# Autodesk Inventor assembly: MechanumChassis
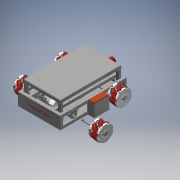
[picture p0: Inventor's stored thumbnail of the model, 180x180]
Saved by Autodesk Inventor 2018 (Build 220112000, 112)
## iProperties
Created: 2017-10-18
Part Number: MechanumChassis
Document SubType Name: Weldment
Designer: Bryce Richards
Mass: 42172.1 g
Surface Area: 44852.8 cm^2
Volume: 5448.29 cm^3
Density: 7.74044 g/cm^3
Weld Material: Steel, Mild, Welded
Author: Bryce Richards
## Documents named in this file (35)
- C:\Users\P136265\Documents\GitHub\mecanum-cad\MechanumChassis.iam
- C:\Users\P136265\Documents\GitHub\mecanum-cad\MecanumFrame2.iam
- C:\Users\P136265\Documents\GitHub\mecanum-cad\PillowAssembly.iam
- C:\Users\P136265\Documents\Inventor\Content Center Files\R2018\en-US\AS 1110\AS 1110 - M8 x 60.ipt
- C:\Users\P136265\Documents\Inventor\Content Center Files\R2018\en-US\AS 1112 (2)\AS 1112 - M8  Type 5.ipt
- C:\Users\P136265\Documents\GitHub\mecanum-cad\PillowPlate.ipt
- C:\Users\P136265\Documents\GitHub\mecanum-cad\LiftPlate.iam
- C:\Users\P136265\Documents\GitHub\mecanum-cad\AlignmentTube.ipt
- C:\Users\P136265\Documents\GitHub\mecanum-cad\WheelShaft.ipt
- C:\Users\P136265\Documents\GitHub\mecanum-cad\Mecanum_Assembly.iam
- C:\Users\P136265\Documents\Inventor\Content Center Files\R2018\en-US\ISO 4032(2)\ISO 4032 - M20 - ISO.ipt
- C:\Users\P136265\Documents\GitHub\mecanum-cad\Cover_FrontRear.ipt
- C:\Users\P136265\Documents\Inventor\Content Center Files\R2018\en-US\CNS 4373\CNS 4373 - M 4.ipt
- C:\Users\P136265\Documents\GitHub\mecanum-cad\Cover_LiftSurface.ipt
- C:\Users\P136265\Documents\GitHub\mecanum-cad\Compressor_PX06.ipt
- C:\Users\P136265\Documents\GitHub\mecanum-cad\RestraintPlate.ipt
- C:\Users\P136265\Documents\Inventor\Content Center Files\R2018\en-US\AS 1420\AS 1420 - 1973 - M4 x 12.ipt
- C:\Users\P136265\Documents\GitHub\mecanum-cad\Cover_Rear.ipt
- C:\Users\P136265\Documents\Inventor\Content Center Files\R2018\en-US\AS 1112 (2)\AS 1112 - M4  Type 5.ipt
- C:\Users\P136265\Documents\Inventor\Content Center Files\R2018\en-US\AS 1110\AS 1110 - M4 x 10.ipt
- C:\Users\P136265\Documents\GitHub\mecanum-cad\LiftBase.ipt
- C:\Users\P136265\Documents\GitHub\mecanum-cad\Firestone.ipt
- C:\Users\P136265\Documents\Inventor\Content Center Files\R2018\en-US\AS 1110\AS 1110 - M8 x 12.ipt
- C:\Users\P136265\Documents\GitHub\mecanum-cad\Nema 23 Stepper Motor Bipolar L=56mm w Gear Ratio 41 Planetary Gearbox.ipt
- C:\Users\P136265\Documents\GitHub\mecanum-cad\Cover_Left.ipt
- C:\Users\P136265\Documents\GitHub\mecanum-cad\Cover_Right.ipt
- C:\Users\P136265\Documents\GitHub\mecanum-cad\BatteryBox_NP1812.ipt
- C:\Users\P136265\Documents\GitHub\mecanum-cad\NP18-12 Battery.ipt
- C:\Users\P136265\Documents\GitHub\mecanum-cad\BearingHousing.iam
- C:\Users\P136265\Documents\mecanum-cad\MechanumChassis\AIP\FEA\cayefugld.fres
- C:\Users\P136265\Documents\mecanum-cad\MechanumChassis\AIP\FEA\cayefugao.fins
- C:\Users\P136265\Documents\mecanum-cad\MechanumChassis\AIP\FEA\cayefugao.fsat
- C:\Users\P136265\Documents\mecanum-cad\MechanumChassis\AIP\FEA\cayefugao.ftes
- C:\Users\P136265\Documents\mecanum-cad\MechanumChassis\AIP\FEA\cayefugao.fwiz
- C:\Users\P136265\Documents\mecanum-cad\MechanumChassis\AIP\FEA\cayefuglc.fmsh
## Components (143 placed, 28 different names)
1. MecanumFrame2:1 [sub-assembly] — Flush:2, Flush:6, Mate:69, Mate:70, Mate:71, Mate:90, Angle:5, Angle:6, Angle:7, Flush:10, Insert:17, Insert:18, Insert:19, Insert:20, Insert:21, Insert:22, Insert:23, Insert:24, Insert:25, Insert:26, Insert:27, Insert:28, Insert:29, Insert:30, Insert:31, Insert:32, Angle:8, Mate:209, Mate:210, Flush:11, Angle:9, Angle:10, Angle:11, Mate:211, Mate:212, Flush:12, Mate:213, Mate:214, Flush:13, Mate:215, Mate:216, Flush:14, Mate:234, Mate:235, Mate:236, Angle:29, Mate:263, Mate:283, Mate:285, Mate:287, Mate:289, Mate:303, Mate:305, Mate:307, Mate:309, Mate:353, Mate:354, Mate:355, Mate:386, Flush:32, Flush:33, Angle:34, Mate:410, Mate:411, Mate:412, Mate:413, Mate:414, Mate:415, Mate:416, Mate:417, Mate:418, Mate:419, Mate:420, Mate:421, Mate:423, Mate:425, Mate:427, Mate:429, Mate:431, Mate:433, Mate:435, Mate:437, Mate:439, Mate:441, Mate:443, Mate:445, Mate:447, Mate:449, Mate:451, Mate:482, Mate:483, Mate:484
2. PillowAssembly:1 [sub-assembly] — Mate:16, Mate:59, Mate:186, Mate:190, Mate:234
3. PillowAssembly:2 [sub-assembly] — Mate:13, Mate:62, Mate:178, Mate:180, Mate:235
4. PillowAssembly:3 [sub-assembly] — Mate:15, Mate:63, Mate:64, Mate:202, Mate:206, Mate:236
5. PillowAssembly:5 [sub-assembly] — Mate:13, Flush:2, Mate:60, Mate:61, Mate:182, Mate:184, Mate:320, Flush:29, Mate:329
6. PillowAssembly:6 [sub-assembly] — Mate:15, Mate:65, Flush:10, Mate:204, Mate:208, Mate:317, Flush:27, Mate:327
7. PillowAssembly:7 [sub-assembly] — Flush:6, Mate:16, Mate:57, Mate:58, Mate:188, Mate:192, Mate:323, Flush:31, Mate:331
8. PillowPlate:2 — Mate:57, Mate:58, Mate:59, Mate:71
9. PillowPlate:3 — Mate:60, Mate:61, Mate:62, Mate:70
10. PillowPlate:4 — Mate:63, Mate:64, Mate:65, Mate:69
11. LiftPlate:1 [sub-assembly] — Angle:29, Angle:30, Angle:31, Angle:32, Angle:33, Mate:263, Mate:311, Flush:22, Flush:23, Mate:413, Mate:414, Mate:481
12. AS 1110 - Metric M8 x 60:33 — Insert:17, Mate:179
13. AS 1110 - Metric M8 x 60:34 — Insert:18, Mate:177
14. AS 1110 - Metric M8 x 60:35 — Insert:19, Mate:183
15. AS 1110 - Metric M8 x 60:36 — Insert:20, Mate:181
16. AS 1110 - Metric M8 x 60:37 — Insert:21, Mate:187
17. AS 1110 - Metric M8 x 60:38 — Insert:22, Mate:191
18. AS 1110 - Metric M8 x 60:39 — Insert:23, Mate:189
19. AS 1110 - Metric M8 x 60:40 — Insert:24, Mate:185
20. AS 1110 - Metric M8 x 60:41 — Insert:25, Mate:199
21. AS 1110 - Metric M8 x 60:42 — Insert:26, Mate:197
22. AS 1110 - Metric M8 x 60:43 — Insert:27, Mate:195
23. AS 1110 - Metric M8 x 60:44 — Insert:28, Mate:193
24. AS 1110 - Metric M8 x 60:45 — Insert:29, Mate:201
25. AS 1110 - Metric M8 x 60:46 — Insert:30, Mate:203
26. AS 1110 - Metric M8 x 60:47 — Insert:31, Mate:207
27. AS 1110 - Metric M8 x 60:48 — Insert:32, Mate:205
28. AS 1112 (2) - Metric M8  Type 5:33 — Mate:177, Mate:178
29. AS 1112 (2) - Metric M8  Type 5:34 — Mate:179, Mate:180
30. AS 1112 (2) - Metric M8  Type 5:35 — Mate:181, Mate:182
31. AS 1112 (2) - Metric M8  Type 5:36 — Mate:183, Mate:184
32. AS 1112 (2) - Metric M8  Type 5:37 — Mate:185, Mate:186
33. AS 1112 (2) - Metric M8  Type 5:38 — Mate:187, Mate:188
34. AS 1112 (2) - Metric M8  Type 5:39 — Mate:189, Mate:190
35. AS 1112 (2) - Metric M8  Type 5:40 — Mate:191, Mate:192
36. AS 1112 (2) - Metric M8  Type 5:41 — Mate:193
37. AS 1112 (2) - Metric M8  Type 5:42 — Mate:195
38. AS 1112 (2) - Metric M8  Type 5:43 — Mate:197
39. AS 1112 (2) - Metric M8  Type 5:44 — Mate:199
40. AS 1112 (2) - Metric M8  Type 5:45 — Mate:201, Mate:202
41. AS 1112 (2) - Metric M8  Type 5:46 — Mate:203, Mate:204
42. AS 1112 (2) - Metric M8  Type 5:47 — Mate:205, Mate:206
43. AS 1112 (2) - Metric M8  Type 5:48 — Mate:207, Mate:208
44. AlignmentTube:1 — Angle:10, Mate:213, Mate:214, Flush:13, Angle:33
45. AlignmentTube:2 — Angle:8, Mate:209, Mate:210, Flush:11, Angle:31
46. AlignmentTube:3 — Angle:11, Mate:215, Mate:216, Flush:14, Angle:32
47. AlignmentTube:4 — Angle:9, Mate:211, Mate:212, Flush:12, Angle:30
48. Mecanum_Assembly:1 [sub-assembly] — Mate:318, Mate:319, Flush:28, Mate:344, Mate:345, Mate:346, Mate:351
49. Mecanum_Assembly:2 [sub-assembly] — Mate:321, Mate:322, Flush:30, Mate:341, Mate:342, Mate:343, Mate:349
50. Mecanum_Assembly:3 [sub-assembly] — Mate:315, Mate:316, Flush:26, Mate:338, Mate:339, Mate:340, Mate:347
51. Mecanum_Assembly:4 [sub-assembly] — Mate:312, Flush:24, Mate:314, Mate:333, Mate:334, Mate:335, Mate:336
52. Cover_FrontRear:1 — Mate:410, Mate:411, Mate:412
53. CNS 4373 M 4:7 — Mate:283
54. CNS 4373 M 4:8 — Mate:285
55. CNS 4373 M 4:9 — Mate:287
56. CNS 4373 M 4:10 — Mate:289
57. CNS 4373 M 4:17 — Mate:303
58. CNS 4373 M 4:18 — Mate:305
59. CNS 4373 M 4:19 — Mate:307
60. CNS 4373 M 4:20 — Mate:309
61. Cover_LiftSurface:1 — Mate:311, Flush:22, Flush:23
62. WheelShaft:1 — Mate:312, Flush:24, Mate:314, Mate:324, Mate:485
63. WheelShaft:2 — Mate:318, Mate:319, Flush:28, Mate:320, Flush:29, Mate:328
64. WheelShaft:3 — Mate:315, Mate:316, Flush:26, Mate:317, Flush:27, Mate:326
65. WheelShaft:4 — Mate:321, Mate:322, Flush:30, Mate:323, Flush:31, Mate:330, Mate:394
66. ISO 4032 M20:1 — Mate:324
67. ISO 4032 M20:2 — Mate:326, Mate:327
68. ISO 4032 M20:3 — Mate:328, Mate:329
69. ISO 4032 M20:4 — Mate:330, Mate:331
70. Compressor_PX06:1 — Mate:356, Mate:358, Mate:367, Mate:368, Mate:369, Mate:370, Mate:371, Mate:372, Mate:373, Mate:374, Mate:375, Mate:376, Mate:377
71. RestraintPlate:1 — Mate:333, Mate:334, Mate:335, Mate:337
72. RestraintPlate:2 — Mate:338, Mate:339, Mate:340, Mate:348
73. RestraintPlate:3 — Mate:341, Mate:342, Mate:343, Mate:350
74. RestraintPlate:4 — Mate:344, Mate:345, Mate:346, Mate:352
75. Cover_Rear:1 — Mate:353, Mate:354, Mate:355, Mate:356, Mate:358, Mate:367, Mate:368, Mate:369, Mate:379, Mate:381, Mate:383, Mate:385
76. AS 1110 - Metric M4 x 10:1 — Mate:370, Mate:371, Mate:378
77. AS 1110 - Metric M4 x 10:2 — Mate:372, Mate:373, Mate:384
78. AS 1110 - Metric M4 x 10:3 — Mate:374, Mate:375, Mate:380
79. AS 1110 - Metric M4 x 10:4 — Mate:376, Mate:377, Mate:382
80. AS 1112 (2) - Metric M4  Type 5:1 — Mate:378, Mate:379
81. AS 1112 (2) - Metric M4  Type 5:2 — Mate:380, Mate:381
82. AS 1112 (2) - Metric M4  Type 5:3 — Mate:382, Mate:383
83. AS 1112 (2) - Metric M4  Type 5:4 — Mate:384, Mate:385
84. LiftBase:1 — Mate:386, Flush:32, Flush:33, Mate:387, Mate:388, Mate:389, Mate:391, Mate:393
85. Firestone:1 — Mate:387, Mate:388, Mate:389, Mate:390, Mate:392, Mate:481
86. AS 1110 - Metric M8 x 12:1 — Mate:390, Mate:391
87. AS 1110 - Metric M8 x 12:2 — Mate:392, Mate:393
88. Nema 23 Stepper Motor Bipolar L=56mm w Gear Ratio 41 Planetary Gearbox:1 — Angle:34, Mate:394
89. Cover_Left:1 — Mate:415, Mate:416, Mate:417, Mate:422, Mate:424, Mate:426, Mate:428, Mate:430, Mate:432, Mate:434, Mate:436, Mate:453, Mate:454, Mate:455, Mate:460, Mate:465, Mate:467, Mate:469, Mate:471
90. Cover_Right:1 — Mate:418, Mate:419, Mate:420, Mate:438, Mate:440, Mate:442, Mate:444, Mate:446, Mate:448, Mate:450, Mate:452, Mate:456, Mate:457, Mate:458, Mate:463, Mate:473, Mate:475, Mate:477, Mate:479
91. CNS 4373 M 4:21 — Mate:421, Mate:422
92. CNS 4373 M 4:22 — Mate:423, Mate:424
93. CNS 4373 M 4:23 — Mate:425, Mate:426
94. CNS 4373 M 4:24 — Mate:427, Mate:428
95. CNS 4373 M 4:25 — Mate:429, Mate:430
96. CNS 4373 M 4:26 — Mate:431, Mate:432
97. CNS 4373 M 4:27 — Mate:433, Mate:434
98. CNS 4373 M 4:28 — Mate:435, Mate:436
99. CNS 4373 M 4:29 — Mate:437, Mate:438
100. CNS 4373 M 4:30 — Mate:439, Mate:440
101. CNS 4373 M 4:31 — Mate:441, Mate:442
102. CNS 4373 M 4:32 — Mate:443, Mate:444
103. CNS 4373 M 4:33 — Mate:445, Mate:446
104. CNS 4373 M 4:34 — Mate:447, Mate:448
105. CNS 4373 M 4:35 — Mate:449, Mate:450
106. CNS 4373 M 4:36 — Mate:451, Mate:452
107. BatteryBox_NP1812:1 — Mate:453, Mate:454, Mate:455, Mate:459, Mate:461, Mate:466, Mate:468, Mate:470, Mate:472
108. BatteryBox_NP1812:2 — Mate:456, Mate:457, Mate:458, Mate:462, Mate:464, Mate:474, Mate:476, Mate:478, Mate:480
109. NP18-12 Battery:1 — Mate:459, Mate:460, Mate:461
110. NP18-12 Battery:2 — Mate:462, Mate:463, Mate:464
111. AS 1112 (2) - Metric M4  Type 5:5 — Mate:465, Mate:466
112. AS 1112 (2) - Metric M4  Type 5:6 — Mate:467, Mate:468
113. AS 1112 (2) - Metric M4  Type 5:7 — Mate:469, Mate:470
114. AS 1112 (2) - Metric M4  Type 5:8 — Mate:471, Mate:472
115. AS 1112 (2) - Metric M4  Type 5:9 — Mate:473, Mate:474
116. AS 1112 (2) - Metric M4  Type 5:10 — Mate:475, Mate:476
117. AS 1112 (2) - Metric M4  Type 5:11 — Mate:477, Mate:478
118. AS 1112 (2) - Metric M4  Type 5:12 — Mate:479, Mate:480
119. BearingHousing:1 [sub-assembly] — Mate:482, Mate:483, Mate:484, Mate:485
120. AS 1420 - Metric M4 x 12:1 — Mate:336, Mate:337
121. AS 1420 - Metric M4 x 12:2
122. AS 1420 - Metric M4 x 12:3
123. AS 1420 - Metric M4 x 12:4
124. AS 1420 - Metric M4 x 12:5
125. AS 1420 - Metric M4 x 12:6
126. AS 1420 - Metric M4 x 12:7 — Mate:347, Mate:348
127. AS 1420 - Metric M4 x 12:8
128. AS 1420 - Metric M4 x 12:9
129. AS 1420 - Metric M4 x 12:10
130. AS 1420 - Metric M4 x 12:11
131. AS 1420 - Metric M4 x 12:12
132. AS 1420 - Metric M4 x 12:13 — Mate:349, Mate:350
133. AS 1420 - Metric M4 x 12:14
134. AS 1420 - Metric M4 x 12:15
135. AS 1420 - Metric M4 x 12:16
136. AS 1420 - Metric M4 x 12:17
137. AS 1420 - Metric M4 x 12:18
138. AS 1420 - Metric M4 x 12:19 — Mate:351, Mate:352
139. AS 1420 - Metric M4 x 12:20
140. AS 1420 - Metric M4 x 12:21
141. AS 1420 - Metric M4 x 12:22
142. AS 1420 - Metric M4 x 12:23
143. AS 1420 - Metric M4 x 12:24
## Component patterns: (6 elements, first: AS 1420 - Metric M4 x 12:1), (6 elements, first: AS 1420 - Metric M4 x 12:7), (6 elements, first: AS 1420 - Metric M4 x 12:13), (6 elements, first: AS 1420 - Metric M4 x 12:19)
## Relationships (259: Mate 212, Flush 18, Insert 16, Angle 13)
- Mate:13: PillowAssembly:2 ↔ PillowAssembly:5
- Flush:2: MecanumFrame2:1 ↔ PillowAssembly:5
- Mate:15: PillowAssembly:3 ↔ PillowAssembly:6
- Flush:6: MecanumFrame2:1 ↔ PillowAssembly:7
- Mate:16: PillowAssembly:1 ↔ PillowAssembly:7
- Mate:57: PillowAssembly:7 ↔ PillowPlate:2
- Mate:58: PillowAssembly:7 ↔ PillowPlate:2
- Mate:59: PillowAssembly:1 ↔ PillowPlate:2
- Mate:60: PillowAssembly:5 ↔ PillowPlate:3
- Mate:61: PillowAssembly:5 ↔ PillowPlate:3
- Mate:62: PillowAssembly:2 ↔ PillowPlate:3
- Mate:63: PillowAssembly:3 ↔ PillowPlate:4
- Mate:64: PillowAssembly:3 ↔ PillowPlate:4
- Mate:65: PillowAssembly:6 ↔ PillowPlate:4
- Mate:69: MecanumFrame2:1 ↔ PillowPlate:4
- Mate:70: MecanumFrame2:1 ↔ PillowPlate:3
- Mate:71: MecanumFrame2:1 ↔ PillowPlate:2
- Mate:90: MecanumFrame2:1
- Angle:5 (0 deg): MecanumFrame2:1
- Angle:6 (0 deg): MecanumFrame2:1
- Angle:7 (0 deg): MecanumFrame2:1
- Flush:10: MecanumFrame2:1 ↔ PillowAssembly:6
- Insert:17: MecanumFrame2:1 ↔ AS 1110 - Metric M8 x 60:33
- Insert:18: MecanumFrame2:1 ↔ AS 1110 - Metric M8 x 60:34
- Insert:19: MecanumFrame2:1 ↔ AS 1110 - Metric M8 x 60:35
- Insert:20: MecanumFrame2:1 ↔ AS 1110 - Metric M8 x 60:36
- Insert:21: MecanumFrame2:1 ↔ AS 1110 - Metric M8 x 60:37
- Insert:22: MecanumFrame2:1 ↔ AS 1110 - Metric M8 x 60:38
- Insert:23: MecanumFrame2:1 ↔ AS 1110 - Metric M8 x 60:39
- Insert:24: MecanumFrame2:1 ↔ AS 1110 - Metric M8 x 60:40
- Insert:25: MecanumFrame2:1 ↔ AS 1110 - Metric M8 x 60:41
- Insert:26: MecanumFrame2:1 ↔ AS 1110 - Metric M8 x 60:42
- Insert:27: MecanumFrame2:1 ↔ AS 1110 - Metric M8 x 60:43
- Insert:28: MecanumFrame2:1 ↔ AS 1110 - Metric M8 x 60:44
- Insert:29: MecanumFrame2:1 ↔ AS 1110 - Metric M8 x 60:45
- Insert:30: MecanumFrame2:1 ↔ AS 1110 - Metric M8 x 60:46
- Insert:31: MecanumFrame2:1 ↔ AS 1110 - Metric M8 x 60:47
- Insert:32: MecanumFrame2:1 ↔ AS 1110 - Metric M8 x 60:48
- Mate:177: AS 1110 - Metric M8 x 60:34 ↔ AS 1112 (2) - Metric M8  Type 5:33
- Mate:178: PillowAssembly:2 ↔ AS 1112 (2) - Metric M8  Type 5:33
- Mate:179: AS 1110 - Metric M8 x 60:33 ↔ AS 1112 (2) - Metric M8  Type 5:34
- Mate:180: PillowAssembly:2 ↔ AS 1112 (2) - Metric M8  Type 5:34
- Mate:181: AS 1110 - Metric M8 x 60:36 ↔ AS 1112 (2) - Metric M8  Type 5:35
- Mate:182: PillowAssembly:5 ↔ AS 1112 (2) - Metric M8  Type 5:35
- Mate:183: AS 1110 - Metric M8 x 60:35 ↔ AS 1112 (2) - Metric M8  Type 5:36
- Mate:184: PillowAssembly:5 ↔ AS 1112 (2) - Metric M8  Type 5:36
- Mate:185: AS 1110 - Metric M8 x 60:40 ↔ AS 1112 (2) - Metric M8  Type 5:37
- Mate:186: PillowAssembly:1 ↔ AS 1112 (2) - Metric M8  Type 5:37
- Mate:187: AS 1110 - Metric M8 x 60:37 ↔ AS 1112 (2) - Metric M8  Type 5:38
- Mate:188: PillowAssembly:7 ↔ AS 1112 (2) - Metric M8  Type 5:38
- Mate:189: AS 1110 - Metric M8 x 60:39 ↔ AS 1112 (2) - Metric M8  Type 5:39
- Mate:190: PillowAssembly:1 ↔ AS 1112 (2) - Metric M8  Type 5:39
- Mate:191: AS 1110 - Metric M8 x 60:38 ↔ AS 1112 (2) - Metric M8  Type 5:40
- Mate:192: PillowAssembly:7 ↔ AS 1112 (2) - Metric M8  Type 5:40
- Mate:193: AS 1110 - Metric M8 x 60:44 ↔ AS 1112 (2) - Metric M8  Type 5:41
- Mate:195: AS 1110 - Metric M8 x 60:43 ↔ AS 1112 (2) - Metric M8  Type 5:42
- Mate:197: AS 1110 - Metric M8 x 60:42 ↔ AS 1112 (2) - Metric M8  Type 5:43
- Mate:199: AS 1110 - Metric M8 x 60:41 ↔ AS 1112 (2) - Metric M8  Type 5:44
- Mate:201: AS 1110 - Metric M8 x 60:45 ↔ AS 1112 (2) - Metric M8  Type 5:45
- Mate:202: PillowAssembly:3 ↔ AS 1112 (2) - Metric M8  Type 5:45
- Mate:203: AS 1110 - Metric M8 x 60:46 ↔ AS 1112 (2) - Metric M8  Type 5:46
- Mate:204: PillowAssembly:6 ↔ AS 1112 (2) - Metric M8  Type 5:46
- Mate:205: AS 1110 - Metric M8 x 60:48 ↔ AS 1112 (2) - Metric M8  Type 5:47
- Mate:206: PillowAssembly:3 ↔ AS 1112 (2) - Metric M8  Type 5:47
- Mate:207: AS 1110 - Metric M8 x 60:47 ↔ AS 1112 (2) - Metric M8  Type 5:48
- Mate:208: PillowAssembly:6 ↔ AS 1112 (2) - Metric M8  Type 5:48
- Angle:8 (0 deg): MecanumFrame2:1 ↔ AlignmentTube:2
- Mate:209: MecanumFrame2:1 ↔ AlignmentTube:2
- Mate:210: MecanumFrame2:1 ↔ AlignmentTube:2
- Flush:11: MecanumFrame2:1 ↔ AlignmentTube:2
- Angle:9 (0 deg): MecanumFrame2:1 ↔ AlignmentTube:4
- Angle:10 (0 deg): MecanumFrame2:1 ↔ AlignmentTube:1
- Angle:11 (0 deg): MecanumFrame2:1 ↔ AlignmentTube:3
- Mate:211: MecanumFrame2:1 ↔ AlignmentTube:4
- Mate:212: MecanumFrame2:1 ↔ AlignmentTube:4
- Flush:12: MecanumFrame2:1 ↔ AlignmentTube:4
- Mate:213: MecanumFrame2:1 ↔ AlignmentTube:1
- Mate:214: MecanumFrame2:1 ↔ AlignmentTube:1
- Flush:13: MecanumFrame2:1 ↔ AlignmentTube:1
- Mate:215: MecanumFrame2:1 ↔ AlignmentTube:3
- Mate:216: MecanumFrame2:1 ↔ AlignmentTube:3
- Flush:14: MecanumFrame2:1 ↔ AlignmentTube:3
- Mate:234: MecanumFrame2:1 ↔ PillowAssembly:1
- Mate:235: MecanumFrame2:1 ↔ PillowAssembly:2
- Mate:236: MecanumFrame2:1 ↔ PillowAssembly:3
- Angle:29 (0 deg): MecanumFrame2:1 ↔ LiftPlate:1
- Angle:30 (0 deg): LiftPlate:1 ↔ AlignmentTube:4
- Angle:31 (0 deg): LiftPlate:1 ↔ AlignmentTube:2
- Angle:32 (0 deg): LiftPlate:1 ↔ AlignmentTube:3
- Angle:33 (0 deg): LiftPlate:1 ↔ AlignmentTube:1
- Mate:263: MecanumFrame2:1 ↔ LiftPlate:1
- Mate:283: MecanumFrame2:1 ↔ CNS 4373 M 4:7
- Mate:285: MecanumFrame2:1 ↔ CNS 4373 M 4:8
- Mate:287: MecanumFrame2:1 ↔ CNS 4373 M 4:9
- Mate:289: MecanumFrame2:1 ↔ CNS 4373 M 4:10
- Mate:303: MecanumFrame2:1 ↔ CNS 4373 M 4:17
- Mate:305: MecanumFrame2:1 ↔ CNS 4373 M 4:18
- Mate:307: MecanumFrame2:1 ↔ CNS 4373 M 4:19
- Mate:309: MecanumFrame2:1 ↔ CNS 4373 M 4:20
- Mate:311: LiftPlate:1 ↔ Cover_LiftSurface:1
- Flush:22 (3 mm): LiftPlate:1 ↔ Cover_LiftSurface:1
- Flush:23 (3 mm): LiftPlate:1 ↔ Cover_LiftSurface:1
- Mate:312: Mecanum_Assembly:4 ↔ WheelShaft:1
- Flush:24: Mecanum_Assembly:4 ↔ WheelShaft:1
- Mate:314: Mecanum_Assembly:4 ↔ WheelShaft:1
- Mate:315: Mecanum_Assembly:3 ↔ WheelShaft:3
- Mate:316: Mecanum_Assembly:3 ↔ WheelShaft:3
- Flush:26: Mecanum_Assembly:3 ↔ WheelShaft:3
- Mate:317: PillowAssembly:6 ↔ WheelShaft:3
- Flush:27 (-25 mm): PillowAssembly:6 ↔ WheelShaft:3
- Mate:318: Mecanum_Assembly:1 ↔ WheelShaft:2
- Mate:319: Mecanum_Assembly:1 ↔ WheelShaft:2
- Flush:28: Mecanum_Assembly:1 ↔ WheelShaft:2
- Mate:320: PillowAssembly:5 ↔ WheelShaft:2
- Flush:29 (-25 mm): PillowAssembly:5 ↔ WheelShaft:2
- Mate:321: Mecanum_Assembly:2 ↔ WheelShaft:4
- Mate:322: Mecanum_Assembly:2 ↔ WheelShaft:4
- Flush:30: Mecanum_Assembly:2 ↔ WheelShaft:4
- Mate:323: PillowAssembly:7 ↔ WheelShaft:4
- Flush:31 (-25 mm): PillowAssembly:7 ↔ WheelShaft:4
- Mate:324: WheelShaft:1 ↔ ISO 4032 M20:1
- Mate:326: WheelShaft:3 ↔ ISO 4032 M20:2
- Mate:327: PillowAssembly:6 ↔ ISO 4032 M20:2
- Mate:328: WheelShaft:2 ↔ ISO 4032 M20:3
- Mate:329: PillowAssembly:5 ↔ ISO 4032 M20:3
- Mate:330: WheelShaft:4 ↔ ISO 4032 M20:4
- Mate:331: PillowAssembly:7 ↔ ISO 4032 M20:4
- Mate:333: Mecanum_Assembly:4 ↔ RestraintPlate:1
- Mate:334: Mecanum_Assembly:4 ↔ RestraintPlate:1
- Mate:335: Mecanum_Assembly:4 ↔ RestraintPlate:1
- Mate:336: Mecanum_Assembly:4 ↔ AS 1420 - Metric M4 x 12:1
- Mate:337: RestraintPlate:1 ↔ AS 1420 - Metric M4 x 12:1
- Mate:338: Mecanum_Assembly:3 ↔ RestraintPlate:2
- Mate:339: Mecanum_Assembly:3 ↔ RestraintPlate:2
- Mate:340: Mecanum_Assembly:3 ↔ RestraintPlate:2
- Mate:341: Mecanum_Assembly:2 ↔ RestraintPlate:3
- Mate:342: Mecanum_Assembly:2 ↔ RestraintPlate:3
- Mate:343: Mecanum_Assembly:2 ↔ RestraintPlate:3
- Mate:344: Mecanum_Assembly:1 ↔ RestraintPlate:4
- Mate:345: Mecanum_Assembly:1 ↔ RestraintPlate:4
- Mate:346: Mecanum_Assembly:1 ↔ RestraintPlate:4
- Mate:347: Mecanum_Assembly:3 ↔ AS 1420 - Metric M4 x 12:7
- Mate:348: RestraintPlate:2 ↔ AS 1420 - Metric M4 x 12:7
- Mate:349: Mecanum_Assembly:2 ↔ AS 1420 - Metric M4 x 12:13
- Mate:350: RestraintPlate:3 ↔ AS 1420 - Metric M4 x 12:13
- Mate:351: Mecanum_Assembly:1 ↔ AS 1420 - Metric M4 x 12:19
- Mate:352: RestraintPlate:4 ↔ AS 1420 - Metric M4 x 12:19
- Mate:353: MecanumFrame2:1 ↔ Cover_Rear:1
- Mate:354: MecanumFrame2:1 ↔ Cover_Rear:1
- Mate:355: MecanumFrame2:1 ↔ Cover_Rear:1
- Mate:356: Compressor_PX06:1 ↔ Cover_Rear:1
- Mate:358: Compressor_PX06:1 ↔ Cover_Rear:1
- Mate:367: Compressor_PX06:1 ↔ Cover_Rear:1
- Mate:368: Compressor_PX06:1 ↔ Cover_Rear:1
- Mate:369: Compressor_PX06:1 ↔ Cover_Rear:1
- Mate:370: Compressor_PX06:1 ↔ AS 1110 - Metric M4 x 10:1
- Mate:371: Compressor_PX06:1 ↔ AS 1110 - Metric M4 x 10:1
- Mate:372: Compressor_PX06:1 ↔ AS 1110 - Metric M4 x 10:2
- Mate:373: Compressor_PX06:1 ↔ AS 1110 - Metric M4 x 10:2
- Mate:374: Compressor_PX06:1 ↔ AS 1110 - Metric M4 x 10:3
- Mate:375: Compressor_PX06:1 ↔ AS 1110 - Metric M4 x 10:3
- Mate:376: Compressor_PX06:1 ↔ AS 1110 - Metric M4 x 10:4
- Mate:377: Compressor_PX06:1 ↔ AS 1110 - Metric M4 x 10:4
- Mate:378: AS 1110 - Metric M4 x 10:1 ↔ AS 1112 (2) - Metric M4  Type 5:1
- Mate:379: Cover_Rear:1 ↔ AS 1112 (2) - Metric M4  Type 5:1
- Mate:380: AS 1110 - Metric M4 x 10:3 ↔ AS 1112 (2) - Metric M4  Type 5:2
- Mate:381: Cover_Rear:1 ↔ AS 1112 (2) - Metric M4  Type 5:2
- Mate:382: AS 1110 - Metric M4 x 10:4 ↔ AS 1112 (2) - Metric M4  Type 5:3
- Mate:383: Cover_Rear:1 ↔ AS 1112 (2) - Metric M4  Type 5:3
- Mate:384: AS 1110 - Metric M4 x 10:2 ↔ AS 1112 (2) - Metric M4  Type 5:4
- Mate:385: Cover_Rear:1 ↔ AS 1112 (2) - Metric M4  Type 5:4
- Mate:386: MecanumFrame2:1 ↔ LiftBase:1
- Flush:32 (2.5 mm): MecanumFrame2:1 ↔ LiftBase:1
- Flush:33 (2.5 mm): MecanumFrame2:1 ↔ LiftBase:1
- Mate:387: LiftBase:1 ↔ Firestone:1
- Mate:388: LiftBase:1 ↔ Firestone:1
- Mate:389: LiftBase:1 ↔ Firestone:1
- Mate:390: Firestone:1 ↔ AS 1110 - Metric M8 x 12:1
- Mate:391: LiftBase:1 ↔ AS 1110 - Metric M8 x 12:1
- Mate:392: Firestone:1 ↔ AS 1110 - Metric M8 x 12:2
- Mate:393: LiftBase:1 ↔ AS 1110 - Metric M8 x 12:2
- Angle:34 (0 deg): MecanumFrame2:1 ↔ Nema 23 Stepper Motor Bipolar L=56mm w Gear Ratio 41 Planetary Gearbox:1
- Mate:394: WheelShaft:4 ↔ Nema 23 Stepper Motor Bipolar L=56mm w Gear Ratio 41 Planetary Gearbox:1
- Mate:410: MecanumFrame2:1 ↔ Cover_FrontRear:1
- Mate:411: MecanumFrame2:1 ↔ Cover_FrontRear:1
- Mate:412: MecanumFrame2:1 ↔ Cover_FrontRear:1
- Mate:413: MecanumFrame2:1 ↔ LiftPlate:1
- Mate:414: MecanumFrame2:1 ↔ LiftPlate:1
- Mate:415: MecanumFrame2:1 ↔ Cover_Left:1
- Mate:416: MecanumFrame2:1 ↔ Cover_Left:1
- Mate:417: MecanumFrame2:1 ↔ Cover_Left:1
- Mate:418: MecanumFrame2:1 ↔ Cover_Right:1
- Mate:419: MecanumFrame2:1 ↔ Cover_Right:1
- Mate:420: MecanumFrame2:1 ↔ Cover_Right:1
- Mate:421: MecanumFrame2:1 ↔ CNS 4373 M 4:21
- Mate:422: Cover_Left:1 ↔ CNS 4373 M 4:21
- Mate:423: MecanumFrame2:1 ↔ CNS 4373 M 4:22
- Mate:424: Cover_Left:1 ↔ CNS 4373 M 4:22
- Mate:425: MecanumFrame2:1 ↔ CNS 4373 M 4:23
- Mate:426: Cover_Left:1 ↔ CNS 4373 M 4:23
- Mate:427: MecanumFrame2:1 ↔ CNS 4373 M 4:24
- Mate:428: Cover_Left:1 ↔ CNS 4373 M 4:24
- Mate:429: MecanumFrame2:1 ↔ CNS 4373 M 4:25
- Mate:430: Cover_Left:1 ↔ CNS 4373 M 4:25
- Mate:431: MecanumFrame2:1 ↔ CNS 4373 M 4:26
- Mate:432: Cover_Left:1 ↔ CNS 4373 M 4:26
- Mate:433: MecanumFrame2:1 ↔ CNS 4373 M 4:27
- Mate:434: Cover_Left:1 ↔ CNS 4373 M 4:27
- Mate:435: MecanumFrame2:1 ↔ CNS 4373 M 4:28
- Mate:436: Cover_Left:1 ↔ CNS 4373 M 4:28
- Mate:437: MecanumFrame2:1 ↔ CNS 4373 M 4:29
- Mate:438: Cover_Right:1 ↔ CNS 4373 M 4:29
- Mate:439: MecanumFrame2:1 ↔ CNS 4373 M 4:30
- Mate:440: Cover_Right:1 ↔ CNS 4373 M 4:30
- Mate:441: MecanumFrame2:1 ↔ CNS 4373 M 4:31
- Mate:442: Cover_Right:1 ↔ CNS 4373 M 4:31
- Mate:443: MecanumFrame2:1 ↔ CNS 4373 M 4:32
- Mate:444: Cover_Right:1 ↔ CNS 4373 M 4:32
- Mate:445: MecanumFrame2:1 ↔ CNS 4373 M 4:33
- Mate:446: Cover_Right:1 ↔ CNS 4373 M 4:33
- Mate:447: MecanumFrame2:1 ↔ CNS 4373 M 4:34
- Mate:448: Cover_Right:1 ↔ CNS 4373 M 4:34
- Mate:449: MecanumFrame2:1 ↔ CNS 4373 M 4:35
- Mate:450: Cover_Right:1 ↔ CNS 4373 M 4:35
- Mate:451: MecanumFrame2:1 ↔ CNS 4373 M 4:36
- Mate:452: Cover_Right:1 ↔ CNS 4373 M 4:36
- Mate:453: Cover_Left:1 ↔ BatteryBox_NP1812:1
- Mate:454: Cover_Left:1 ↔ BatteryBox_NP1812:1
- Mate:455: Cover_Left:1 ↔ BatteryBox_NP1812:1
- Mate:456: Cover_Right:1 ↔ BatteryBox_NP1812:2
- Mate:457: Cover_Right:1 ↔ BatteryBox_NP1812:2
- Mate:458: Cover_Right:1 ↔ BatteryBox_NP1812:2
- Mate:459: BatteryBox_NP1812:1 ↔ NP18-12 Battery:1
- Mate:460 (2 mm): Cover_Left:1 ↔ NP18-12 Battery:1
- Mate:461 (2 mm): BatteryBox_NP1812:1 ↔ NP18-12 Battery:1
- Mate:462: BatteryBox_NP1812:2 ↔ NP18-12 Battery:2
- Mate:463 (2 mm): Cover_Right:1 ↔ NP18-12 Battery:2
- Mate:464 (2 mm): BatteryBox_NP1812:2 ↔ NP18-12 Battery:2
- Mate:465: Cover_Left:1 ↔ AS 1112 (2) - Metric M4  Type 5:5
- Mate:466: BatteryBox_NP1812:1 ↔ AS 1112 (2) - Metric M4  Type 5:5
- Mate:467: Cover_Left:1 ↔ AS 1112 (2) - Metric M4  Type 5:6
- Mate:468: BatteryBox_NP1812:1 ↔ AS 1112 (2) - Metric M4  Type 5:6
- Mate:469: Cover_Left:1 ↔ AS 1112 (2) - Metric M4  Type 5:7
- Mate:470: BatteryBox_NP1812:1 ↔ AS 1112 (2) - Metric M4  Type 5:7
- Mate:471: Cover_Left:1 ↔ AS 1112 (2) - Metric M4  Type 5:8
- Mate:472: BatteryBox_NP1812:1 ↔ AS 1112 (2) - Metric M4  Type 5:8
- Mate:473: Cover_Right:1 ↔ AS 1112 (2) - Metric M4  Type 5:9
- Mate:474: BatteryBox_NP1812:2 ↔ AS 1112 (2) - Metric M4  Type 5:9
- Mate:475: Cover_Right:1 ↔ AS 1112 (2) - Metric M4  Type 5:10
- Mate:476: BatteryBox_NP1812:2 ↔ AS 1112 (2) - Metric M4  Type 5:10
- Mate:477: Cover_Right:1 ↔ AS 1112 (2) - Metric M4  Type 5:11
- Mate:478: BatteryBox_NP1812:2 ↔ AS 1112 (2) - Metric M4  Type 5:11
- Mate:479: Cover_Right:1 ↔ AS 1112 (2) - Metric M4  Type 5:12
- Mate:480: BatteryBox_NP1812:2 ↔ AS 1112 (2) - Metric M4  Type 5:12
- Mate:481: LiftPlate:1 ↔ Firestone:1
- Mate:482: MecanumFrame2:1 ↔ BearingHousing:1
- Mate:483: MecanumFrame2:1 ↔ BearingHousing:1
- Mate:484: MecanumFrame2:1 ↔ BearingHousing:1
- Mate:485: WheelShaft:1 ↔ BearingHousing:1
## Named parameters: sa_0 = 0, sa_1 = -3.88819e-08, sa_2 = 1e+06
note: some values were not read from the file. Shown as the stored number, unit unknown: "sa_0", "sa_1", "sa_2".
